# Autodesk Inventor assembly: Teljes
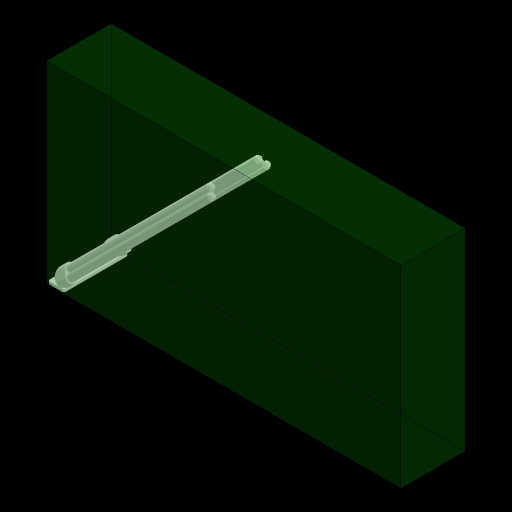
[picture p0: Inventor's stored thumbnail of the model, 512x512]
Saved by Autodesk Inventor 2023 (Build 270158000, 158)
## iProperties
Created: 2022-11-09
Part Number: Teljes
Document SubType Name: Assembly
Designer: gd1
Author: gd1
## Documents named in this file (4)
- C:\Users\gd1\3D Objects\3D nagyteherbírású híd\hid\Teljes.iam
- C:\Users\gd1\3D Objects\3D nagyteherbírású híd\hid\45 fok középre.ipt
- C:\Users\gd1\3D Objects\3D nagyteherbírású híd\hid\palca 325mm.ipt
- C:\Users\gd1\3D Objects\3D nagyteherbírású híd\hid\Part3.ipt
## Components (4 placed, 3 different names)
1. 45 fok középre:1 — Rotational:1, Rotational:2
2. palca 325mm:1 — Rotational:1
3. palca 325mm:2 — Rotational:2
4. Part3:1
## Relationships (2: RevoluteJoint 2)
- Rotational:1 [RevoluteJoint]: 45 fok középre:1 ↔ palca 325mm:1
- Rotational:2 [RevoluteJoint]: 45 fok középre:1 ↔ palca 325mm:2
